# Autodesk Inventor assembly: derive_rod_v7
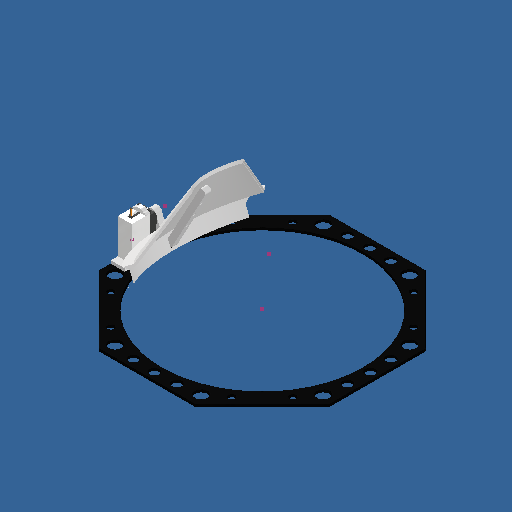
[picture p0: Inventor's stored thumbnail of the model, 512x512]
Saved by Autodesk Inventor 2026.2 (Build 302298000, 298)
## iProperties
Created: 2026-01-13
Part Number: derive_rod_v7
Document SubType Name: Assembly
Designer: Thoma
Author: Thoma
## Documents named in this file (6)
- C:\Users\Thoma\OneDrive\Desktop\dir\telescope_cover\cover\derive_rod_v10.iam
- C:\Users\Thoma\OneDrive\Desktop\dir\telescope_cover\telescope\version_3\Telescope_End.ipt
- C:\Users\Thoma\OneDrive\Desktop\dir\telescope_cover\cover\Cover_Upper_v3.ipt
- C:\Users\Thoma\OneDrive\Desktop\dir\telescope_cover\servo\DSS-M15S Servo.ipt
- C:\Users\Thoma\OneDrive\Desktop\dir\telescope_cover\cover\rod_v9.ipt
- C:\Users\Thoma\OneDrive\Desktop\dir\telescope_cover\cover\base+casing_v1.ipt
## Components (5 placed, 5 different names)
1. Telescope_End:1 — Flush:1, Mate:12, Mate:13, Mate:14
2. Cover_Upper_v3:1 — Mate:7, Mate:8, Tangent:1
3. DSS-M15S Servo:1 — Flush:1, Mate:10, Mate:11, Mate:15, Mate:16, Mate:17
4. rod_v9:1 — Mate:7, Mate:8, Tangent:1, Mate:10, Mate:11
5. base+casing_v1:1 — Mate:12, Mate:13, Mate:14, Mate:15, Mate:16, Mate:17
## Relationships (12: Mate 10, Flush 1, Tangent 1)
- Flush:1 (2.5 mm): Telescope_End:1 ↔ DSS-M15S Servo:1
- Mate:7: Cover_Upper_v3:1 ↔ rod_v9:1
- Mate:8: Cover_Upper_v3:1 ↔ rod_v9:1
- Tangent:1 (-1 mm): Cover_Upper_v3:1 ↔ rod_v9:1
- Mate:10 (0.57 mm): DSS-M15S Servo:1 ↔ rod_v9:1
- Mate:11: DSS-M15S Servo:1 ↔ rod_v9:1
- Mate:12: Telescope_End:1 ↔ base+casing_v1:1
- Mate:13: Telescope_End:1 ↔ base+casing_v1:1
- Mate:14: Telescope_End:1 ↔ base+casing_v1:1
- Mate:15 (0.1 mm): DSS-M15S Servo:1 ↔ base+casing_v1:1
- Mate:16 (1.1 mm): DSS-M15S Servo:1 ↔ base+casing_v1:1
- Mate:17: DSS-M15S Servo:1 ↔ base+casing_v1:1
